# Autodesk Inventor assembly: 全身
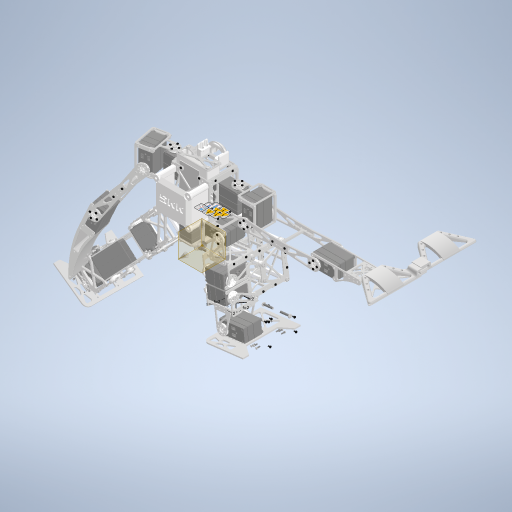
[picture p0: Inventor's stored thumbnail of the model, 512x512]
Saved by Autodesk Inventor 2024 (Build 280153000, 153)
## iProperties
Created: 2023-03-27
Part Number: 全身
Document SubType Name: Assembly
Designer: right
Mass: 1068.94 g
Surface Area: 4163.89 cm^2
Volume: 624.673 cm^3
Density: 1.71121 g/cm^3
Author: right
## Documents named in this file (11)
- C:\Users\right\OneDrive\ドキュメント\Inventor\V2二足Light＿仮\全身.iam
- C:\Users\right\OneDrive\ドキュメント\Inventor\V2二足Light＿仮\kosi.iam
- C:\Users\right\OneDrive\ドキュメント\Inventor\V2二足Light＿仮\足.iam
- C:\Users\right\OneDrive\ドキュメント\Inventor\V2二足Light＿仮\上半身.iam
- C:\Users\right\OneDrive\ドキュメント\Inventor\V2二足Light＿仮\足2.iam
- C:\Users\right\OneDrive\ドキュメント\Inventor\V2二足Light＿仮\spacer.ipt
- C:\Users\right\OneDrive\ドキュメント\Inventor\V2二足Light＿仮\spacer1.ipt
- C:\Users\right\OneDrive\ドキュメント\Inventor\V2二足Light＿仮\M3中ねじ.ipt
- C:\Users\right\OneDrive\ドキュメント\Inventor\V2二足Light＿仮\M3長ねじ.ipt
- C:\Users\right\OneDrive\ドキュメント\Inventor\V2二足Light＿仮\M3長ねじ_MIR.ipt
- C:\Users\right\OneDrive\ドキュメント\Inventor\V2二足Light＿仮\M3中ねじ_MIR.ipt
## Components (62 placed, 10 different names)
1. kosi:1 [sub-assembly] — 挿入:2, 挿入:7, 角度:1, 挿入:8
2. 足:1 [sub-assembly] — 挿入:2, 挿入:9, 挿入:10, 挿入:11, 挿入:12, 挿入:13, 挿入:14, 挿入:15, 挿入:16, 挿入:25, 挿入:26, 挿入:27, 挿入:28, 挿入:29, 挿入:30, 挿入:31, 挿入:32, 挿入:33, 挿入:34, 挿入:48, 挿入:49, 挿入:50, 挿入:53, 挿入:73
3. 上半身:1 [sub-assembly] — 挿入:7, 角度:1, 挿入:58, 挿入:59, 挿入:61, 挿入:62, 挿入:63, 挿入:64, 挿入:65, 挿入:66, メイト:1, 挿入:68, 挿入:69, 挿入:70, 挿入:71, 挿入:72
4. 足2:1 [sub-assembly] — 挿入:8, 挿入:17, 挿入:18, 挿入:19, 挿入:20, 挿入:21, 挿入:22, 挿入:35, 挿入:36, 挿入:37, 挿入:38, 挿入:39, 挿入:40, 挿入:41, 挿入:42, 挿入:43, 挿入:44, 挿入:45, 挿入:46, 挿入:47, 挿入:54, 挿入:55, 挿入:56, 挿入:57
5. spacer:1 — 挿入:11, 挿入:12
6. spacer:2 — 挿入:9, 挿入:10
7. spacer:3 — 挿入:14
8. spacer:4 — 挿入:13
9. spacer:5 — 挿入:15
10. spacer:6 — 挿入:16
11. spacer1:1 — 挿入:21
12. spacer1:2 — 挿入:18
13. spacer1:3 — 挿入:20
14. spacer1:4 — 挿入:19
15. spacer1:5 — 挿入:22
16. spacer1:6 — 挿入:17
17. M3長ねじ:1
18. M3長ねじ:2 — 挿入:73
19. M3長ねじ:3 — 挿入:25
20. M3長ねじ:4 — 挿入:26
21. M3長ねじ:5 — 挿入:27
22. M3長ねじ:6 — 挿入:28
23. M3長ねじ:7 — 挿入:29
24. M3長ねじ:8 — 挿入:30
25. M3長ねじ:9 — 挿入:31
26. M3長ねじ:10 — 挿入:32
27. M3長ねじ:11 — 挿入:33
28. M3長ねじ:12 — 挿入:34
29. M3長ねじ_MIR:1 — 挿入:36
30. M3長ねじ_MIR:2 — 挿入:35, 挿入:47
31. M3長ねじ_MIR:3 — 挿入:37
32. M3長ねじ_MIR:4 — 挿入:46
33. M3長ねじ_MIR:5 — 挿入:38
34. M3長ねじ_MIR:6 — 挿入:45
35. M3長ねじ_MIR:7 — 挿入:44
36. M3長ねじ_MIR:8 — 挿入:43
37. M3長ねじ_MIR:9 — 挿入:40
38. M3長ねじ_MIR:10 — 挿入:39
39. M3長ねじ_MIR:11 — 挿入:41
40. M3長ねじ_MIR:12 — 挿入:42
41. M3中ねじ:1 — 挿入:48
42. M3中ねじ:2 — 挿入:49
43. M3中ねじ:3 — 挿入:50
44. M3中ねじ:6 — 挿入:53
45. M3中ねじ_MIR:1 — 挿入:54
46. M3中ねじ_MIR:2 — 挿入:55
47. M3中ねじ_MIR:3 — 挿入:56
48. M3中ねじ_MIR:4 — 挿入:59
49. M3中ねじ_MIR:5 — 挿入:58
50. M3中ねじ_MIR:6 — 挿入:57
51. M3中ねじ_MIR:7 — 挿入:61
52. M3中ねじ:8 — 挿入:62
53. M3中ねじ:9 — 挿入:63
54. M3中ねじ:10 — 挿入:64
55. M3中ねじ:11 — 挿入:65, 挿入:67
56. M3中ねじ:12 — 挿入:66
57. M3中ねじ:13 — メイト:1, 挿入:67
58. M3中ねじ_MIR:8 — 挿入:68
59. M3中ねじ_MIR:9 — 挿入:69
60. M3中ねじ_MIR:10 — 挿入:70
61. M3中ねじ:14 — 挿入:71
62. M3中ねじ:15 — 挿入:72
## Relationships (65: Insert 63, Angle 1, Mate 1)
- 挿入:2 [Insert]: kosi:1 ↔ 足:1
- 挿入:7 [Insert]: kosi:1 ↔ 上半身:1
- 角度:1 [Angle] (0 deg): kosi:1 ↔ 上半身:1
- 挿入:8 [Insert]: kosi:1 ↔ 足2:1
- 挿入:9 [Insert]: 足:1 ↔ spacer:2
- 挿入:10 [Insert]: 足:1 ↔ spacer:2
- 挿入:11 [Insert]: 足:1 ↔ spacer:1
- 挿入:12 [Insert]: 足:1 ↔ spacer:1
- 挿入:13 [Insert]: 足:1 ↔ spacer:4
- 挿入:14 [Insert]: 足:1 ↔ spacer:3
- 挿入:15 [Insert]: 足:1 ↔ spacer:5
- 挿入:16 [Insert]: 足:1 ↔ spacer:6
- 挿入:17 [Insert]: 足2:1 ↔ spacer1:6
- 挿入:18 [Insert]: 足2:1 ↔ spacer1:2
- 挿入:19 [Insert]: 足2:1 ↔ spacer1:4
- 挿入:20 [Insert]: 足2:1 ↔ spacer1:3
- 挿入:21 [Insert]: 足2:1 ↔ spacer1:1
- 挿入:22 [Insert]: 足2:1 ↔ spacer1:5
- 挿入:25 [Insert]: 足:1 ↔ M3長ねじ:3
- 挿入:26 [Insert]: 足:1 ↔ M3長ねじ:4
- 挿入:27 [Insert]: 足:1 ↔ M3長ねじ:5
- 挿入:28 [Insert]: 足:1 ↔ M3長ねじ:6
- 挿入:29 [Insert]: 足:1 ↔ M3長ねじ:7
- 挿入:30 [Insert]: 足:1 ↔ M3長ねじ:8
- 挿入:31 [Insert]: 足:1 ↔ M3長ねじ:9
- 挿入:32 [Insert]: 足:1 ↔ M3長ねじ:10
- 挿入:33 [Insert]: 足:1 ↔ M3長ねじ:11
- 挿入:34 [Insert]: 足:1 ↔ M3長ねじ:12
- 挿入:35 [Insert]: 足2:1 ↔ M3長ねじ_MIR:2
- 挿入:36 [Insert]: 足2:1 ↔ M3長ねじ_MIR:1
- 挿入:37 [Insert]: 足2:1 ↔ M3長ねじ_MIR:3
- 挿入:38 [Insert]: 足2:1 ↔ M3長ねじ_MIR:5
- 挿入:39 [Insert]: 足2:1 ↔ M3長ねじ_MIR:10
- 挿入:40 [Insert]: 足2:1 ↔ M3長ねじ_MIR:9
- 挿入:41 [Insert]: 足2:1 ↔ M3長ねじ_MIR:11
- 挿入:42 [Insert]: 足2:1 ↔ M3長ねじ_MIR:12
- 挿入:43 [Insert]: 足2:1 ↔ M3長ねじ_MIR:8
- 挿入:44 [Insert]: 足2:1 ↔ M3長ねじ_MIR:7
- 挿入:45 [Insert]: 足2:1 ↔ M3長ねじ_MIR:6
- 挿入:46 [Insert]: 足2:1 ↔ M3長ねじ_MIR:4
- 挿入:47 [Insert]: 足2:1 ↔ M3長ねじ_MIR:2
- 挿入:48 [Insert]: 足:1 ↔ M3中ねじ:1
- 挿入:49 [Insert]: 足:1 ↔ M3中ねじ:2
- 挿入:50 [Insert]: 足:1 ↔ M3中ねじ:3
- 挿入:53 [Insert]: 足:1 ↔ M3中ねじ:6
- 挿入:54 [Insert]: 足2:1 ↔ M3中ねじ_MIR:1
- 挿入:55 [Insert]: 足2:1 ↔ M3中ねじ_MIR:2
- 挿入:56 [Insert]: 足2:1 ↔ M3中ねじ_MIR:3
- 挿入:57 [Insert]: 足2:1 ↔ M3中ねじ_MIR:6
- 挿入:58 [Insert]: 上半身:1 ↔ M3中ねじ_MIR:5
- 挿入:59 [Insert]: 上半身:1 ↔ M3中ねじ_MIR:4
- 挿入:61 [Insert]: 上半身:1 ↔ M3中ねじ_MIR:7
- 挿入:62 [Insert]: 上半身:1 ↔ M3中ねじ:8
- 挿入:63 [Insert]: 上半身:1 ↔ M3中ねじ:9
- 挿入:64 [Insert]: 上半身:1 ↔ M3中ねじ:10
- 挿入:65 [Insert]: 上半身:1 ↔ M3中ねじ:11
- 挿入:66 [Insert]: 上半身:1 ↔ M3中ねじ:12
- メイト:1 [Mate]: 上半身:1 ↔ M3中ねじ:13
- 挿入:67 [Insert] (1 mm): M3中ねじ:11 ↔ M3中ねじ:13
- 挿入:68 [Insert]: 上半身:1 ↔ M3中ねじ_MIR:8
- 挿入:69 [Insert]: 上半身:1 ↔ M3中ねじ_MIR:9
- 挿入:70 [Insert]: 上半身:1 ↔ M3中ねじ_MIR:10
- 挿入:71 [Insert]: 上半身:1 ↔ M3中ねじ:14
- 挿入:72 [Insert]: 上半身:1 ↔ M3中ねじ:15
- 挿入:73 [Insert]: 足:1 ↔ M3長ねじ:2
